# Autodesk Inventor assembly: Motor Shaft
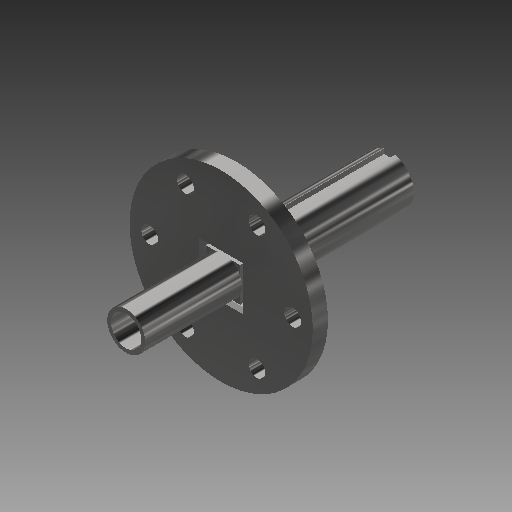
[picture p0: Inventor's stored thumbnail of the model, 512x512]
Saved by Autodesk Inventor 2019 (Build 230136000, 136)
## iProperties
Created: 2018-11-07
Part Number: Motor Shaft
Document SubType Name: Assembly
Designer: robinsat
Description: Revised Motor Shaft
Mass: 574.176 g
Surface Area: 334.337 cm^2
Volume: 118.928 cm^3
Density: 4.82792 g/cm^3
Material_size: Provided Motor Shaft
Quantity: 1
Author: Adam Robinson
Title: Motor Shaft Modification
## Documents named in this file (3)
- P:\me_fsae\2018_2019\ME\DriveTrain\Dyno\Adam'sMotorShaftV3.iam
- P:\me_fsae\2018_2019\ME\DriveTrain\Dyno\Adam's Motor Shaft Rev2.ipt
- P:\me_fsae\2018_2019\ME\DriveTrain\Dyno\Adam's Shaft plate rev 2.ipt
## Components (2 placed, 2 different names)
1. Adam's Motor Shaft Rev2:1 — Mate:1, Mate:2, Mate:3
2. Adam's Shaft plate rev 2:1 — Mate:1, Mate:2, Mate:3
## Relationships (3: Mate 3)
- Mate:1: Adam's Motor Shaft Rev2:1 ↔ Adam's Shaft plate rev 2:1
- Mate:2: Adam's Motor Shaft Rev2:1 ↔ Adam's Shaft plate rev 2:1
- Mate:3: Adam's Motor Shaft Rev2:1 ↔ Adam's Shaft plate rev 2:1
